# Autodesk Inventor assembly: Winch MK4
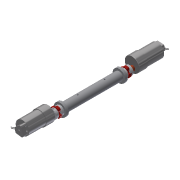
[picture p0: Inventor's stored thumbnail of the model, 180x180]
Saved by Autodesk Inventor 2013 (Build 170138000, 138)
## iProperties
Created: 2014-01-06
Part Number: Winch MK4
Document SubType Name: Assembly
Designer: kahohbein
Author: kahohbein
## Documents named in this file (6)
- C:\Users\nojessen\Documents\GitHub\2013-2014_BlockParty\CAD\Lift\MK4\Winch MK4.iam
- C:\Users\nojessen\Documents\GitHub\2013-2014_BlockParty\CAD\Lift\MK4\custom pvc spool.ipt
- C:\Users\nojessen\Documents\GitHub\2013-2014_BlockParty\CAD\Lift\MK4\end piece for spool.ipt
- C:\Users\nojessen\Documents\GitHub\2013-2014_BlockParty\CAD\COTSParts\Tetrix\Tetrix hub - motor.ipt
- C:\Users\nojessen\Documents\GitHub\2013-2014_BlockParty\CAD\COTSParts\Tetrix\Tetrix motor.ipt
- C:\Users\nojessen\Documents\GitHub\2013-2014_BlockParty\CAD\delete me\Part6.ipt
## Components (11 placed, 5 different names)
1. custom pvc spool:1 — Mate:1, Mate:4, Mate:25, Mate:38, Mate:42, Mate:43
2. end piece for spool:1 — Mate:1, Mate:37, Mate:41, Mate:42
3. end piece for spool:2 — Mate:4, Mate:35, Mate:38, Mate:43
4. Tetrix motor:1 — Mate:15, Mate:29, Mate:30, Mate:32
5. Tetrix motor:2 — Mate:15, Mate:22, Mate:23, Mate:25, Mate:34
6. Part6:1 — Mate:26, Mate:27, Mate:28, Mate:31
7. Part6:2 — Mate:18, Mate:19, Mate:24, Mate:33
8. Tetrix hub - motor:4 — Mate:18, Mate:19, Mate:22, Mate:23, Mate:24
9. Tetrix hub - motor:5 — Mate:26, Mate:27, Mate:28, Mate:29, Mate:30
10. Tetrix hub - motor:6 — Mate:33, Mate:34, Mate:35
11. Tetrix hub - motor:7 — Mate:31, Mate:32, Mate:37, Mate:41
## Relationships (24: Mate 24)
- Mate:1: custom pvc spool:1 ↔ end piece for spool:1
- Mate:4: custom pvc spool:1 ↔ end piece for spool:2
- Mate:15: Tetrix motor:1 ↔ Tetrix motor:2
- Mate:18: Part6:2 ↔ Tetrix hub - motor:4
- Mate:19: Part6:2 ↔ Tetrix hub - motor:4
- Mate:22: Tetrix motor:2 ↔ Tetrix hub - motor:4
- Mate:23: Tetrix motor:2 ↔ Tetrix hub - motor:4
- Mate:24: Part6:2 ↔ Tetrix hub - motor:4
- Mate:25: custom pvc spool:1 ↔ Tetrix motor:2
- Mate:26: Part6:1 ↔ Tetrix hub - motor:5
- Mate:27: Part6:1 ↔ Tetrix hub - motor:5
- Mate:28: Part6:1 ↔ Tetrix hub - motor:5
- Mate:29: Tetrix motor:1 ↔ Tetrix hub - motor:5
- Mate:30: Tetrix motor:1 ↔ Tetrix hub - motor:5
- Mate:31: Part6:1 ↔ Tetrix hub - motor:7
- Mate:32: Tetrix motor:1 ↔ Tetrix hub - motor:7
- Mate:33: Part6:2 ↔ Tetrix hub - motor:6
- Mate:34: Tetrix motor:2 ↔ Tetrix hub - motor:6
- Mate:35: end piece for spool:2 ↔ Tetrix hub - motor:6
- Mate:37: end piece for spool:1 ↔ Tetrix hub - motor:7
- Mate:38: custom pvc spool:1 ↔ end piece for spool:2
- Mate:41: end piece for spool:1 ↔ Tetrix hub - motor:7
- Mate:42: custom pvc spool:1 ↔ end piece for spool:1
- Mate:43: custom pvc spool:1 ↔ end piece for spool:2
